# Autodesk Inventor assembly: UpperArm
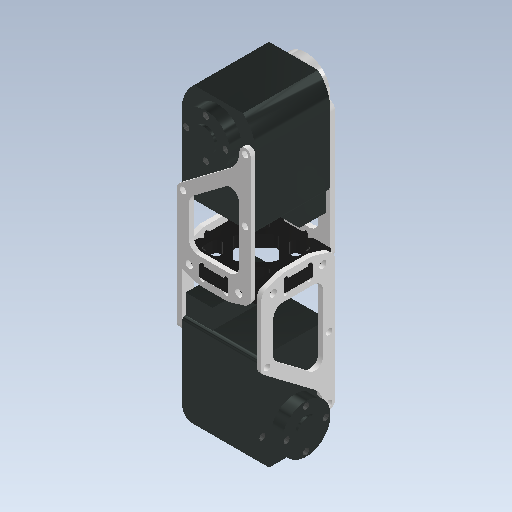
[picture p0: Inventor's stored thumbnail of the model, 512x512]
Saved by Autodesk Inventor 2020.4 (Build 244396000, 396)
## iProperties
Created: 2021-09-11
Part Number: UpperArm
Document SubType Name: Assembly
Designer: Masato
Author: Masato
## Documents named in this file (6)
- C:\Users\Masato\Documents\Inventor\CIT Brains_Inventor\OpenPlatform_ver3_0\UpperBody\Arm\UpperArm.iam
- C:\Users\Masato\Documents\Inventor\CIT Brains_Inventor\OpenPlatform_ver3_0\UpperBody\Arm\UpperArm_vertical_frame_01.ipt
- C:\Users\Masato\Documents\Inventor\CIT Brains_Inventor\OpenPlatform_ver3_0\UpperBody\Arm\UpperArm_horizontal_frame_01.ipt
- C:\Users\Masato\Documents\Inventor\CIT Brains_Inventor\OpenPlatform_ver3_0\Ready_Made\B3M10xx.ipt
- B3M11xx.ipt
- C:\Users\Masato\Documents\Inventor\CIT Brains_Inventor\OpenPlatform_ver3_0\Ready_Made\free_horn.ipt
## Components (9 placed, 4 different names)
1. UpperArm_horizontal_frame_01:1 — 挿入:7, 挿入:8, 挿入:9, 挿入:10, 挿入:11, 挿入:12, 挿入:13, 挿入:14
2. UpperArm_vertical_frame_01:1 — 挿入:1, 挿入:2, 挿入:3, 挿入:7, 挿入:8
3. UpperArm_vertical_frame_01:2 — 挿入:4, 挿入:5, 挿入:6, 挿入:9, 挿入:10
4. UpperArm_vertical_frame_01:3 — 挿入:11, 挿入:12, 挿入:15, 挿入:16, 挿入:17
5. UpperArm_vertical_frame_01:4 — 挿入:13, 挿入:14, 挿入:18, 挿入:19, 挿入:20
6. B3M10xx:1 — 挿入:1, 挿入:2, 挿入:3, 挿入:4, 挿入:5, 挿入:6, 挿入:22
7. B3M10xx:2 — 挿入:15, 挿入:16, 挿入:17, 挿入:18, 挿入:19, 挿入:20, 挿入:21
8. free_horn:1 — 挿入:22
9. free_horn:2 — 挿入:21
## Relationships (22: Insert 22)
- 挿入:1 [Insert]: UpperArm_vertical_frame_01:1 ↔ B3M10xx:1
- 挿入:2 [Insert]: UpperArm_vertical_frame_01:1 ↔ B3M10xx:1
- 挿入:3 [Insert]: UpperArm_vertical_frame_01:1 ↔ B3M10xx:1
- 挿入:4 [Insert]: UpperArm_vertical_frame_01:2 ↔ B3M10xx:1
- 挿入:5 [Insert]: UpperArm_vertical_frame_01:2 ↔ B3M10xx:1
- 挿入:6 [Insert]: UpperArm_vertical_frame_01:2 ↔ B3M10xx:1
- 挿入:7 [Insert]: UpperArm_horizontal_frame_01:1 ↔ UpperArm_vertical_frame_01:1
- 挿入:8 [Insert]: UpperArm_horizontal_frame_01:1 ↔ UpperArm_vertical_frame_01:1
- 挿入:9 [Insert]: UpperArm_horizontal_frame_01:1 ↔ UpperArm_vertical_frame_01:2
- 挿入:10 [Insert]: UpperArm_horizontal_frame_01:1 ↔ UpperArm_vertical_frame_01:2
- 挿入:11 [Insert]: UpperArm_horizontal_frame_01:1 ↔ UpperArm_vertical_frame_01:3
- 挿入:12 [Insert]: UpperArm_horizontal_frame_01:1 ↔ UpperArm_vertical_frame_01:3
- 挿入:13 [Insert]: UpperArm_horizontal_frame_01:1 ↔ UpperArm_vertical_frame_01:4
- 挿入:14 [Insert]: UpperArm_horizontal_frame_01:1 ↔ UpperArm_vertical_frame_01:4
- 挿入:15 [Insert]: UpperArm_vertical_frame_01:3 ↔ B3M10xx:2
- 挿入:16 [Insert]: UpperArm_vertical_frame_01:3 ↔ B3M10xx:2
- 挿入:17 [Insert]: UpperArm_vertical_frame_01:3 ↔ B3M10xx:2
- 挿入:18 [Insert]: UpperArm_vertical_frame_01:4 ↔ B3M10xx:2
- 挿入:19 [Insert]: UpperArm_vertical_frame_01:4 ↔ B3M10xx:2
- 挿入:20 [Insert]: UpperArm_vertical_frame_01:4 ↔ B3M10xx:2
- 挿入:21 [Insert]: B3M10xx:2 ↔ free_horn:2
- 挿入:22 [Insert]: B3M10xx:1 ↔ free_horn:1
